# Autodesk Inventor assembly: LJ12A3-4-Z-BY
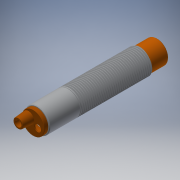
[picture p0: Inventor's stored thumbnail of the model, 180x180]
Saved by Autodesk Inventor 2016 SP1 (Build 200210100, 210)
## iProperties
Created: 2014-03-08
Part Number: LJ12A3-4-Z-BY
Document SubType Name: Assembly
Designer: PowerStation9000
Sending System: SolidWorks 2011
Last Author: i.miroslavov
Last Saved: 2014-03-08
Author: PowerStation9000
## Documents named in this file (4)
- C:\Users\PowerStation9000\AppData\Local\Autodesk\Autodesk Sync\Cloud\mathiaslk\UltiBot mk2\Importerede komponenter\Proxy probe\LJ12A3-4-Z-BY.iam
- C:\Users\PowerStation9000\AppData\Local\Autodesk\Autodesk Sync\Cloud\mathiaslk\UltiBot mk2\Importerede komponenter\Proxy probe\LJ12A3-4-Z-BY-1.ipt
- C:\Users\PowerStation9000\AppData\Local\Autodesk\Autodesk Sync\Cloud\mathiaslk\UltiBot mk2\Importerede komponenter\Proxy probe\LJ12A3-4-Z-BY-2.ipt
- C:\Users\PowerStation9000\AppData\Local\Autodesk\Autodesk Sync\Cloud\mathiaslk\UltiBot mk2\Importerede komponenter\Proxy probe\LJ12A3-4-Z-BY-3.ipt
## Components (3 placed, 3 different names)
1. LJ12A3-4-Z-BY-1:1 — Mate:1, Mate:6, Mate:7, Mate:8
2. LJ12A3-4-Z-BY-2:2 — Mate:6, Mate:7
3. LJ12A3-4-Z-BY-3:1 — Mate:1, Mate:8
## Relationships (4: Mate 4)
- Mate:1: LJ12A3-4-Z-BY-1:1 ↔ LJ12A3-4-Z-BY-3:1
- Mate:6: LJ12A3-4-Z-BY-1:1 ↔ LJ12A3-4-Z-BY-2:2
- Mate:7: LJ12A3-4-Z-BY-1:1 ↔ LJ12A3-4-Z-BY-2:2
- Mate:8: LJ12A3-4-Z-BY-1:1 ↔ LJ12A3-4-Z-BY-3:1
